# Autodesk Inventor assembly: Longhouse
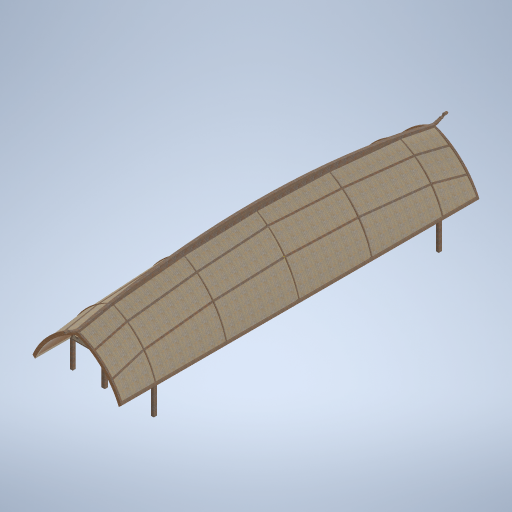
[picture p0: Inventor's stored thumbnail of the model, 512x512]
Saved by Autodesk Inventor 2024.2 (Build 282272000, 272)
## iProperties
Created: 2024-05-22
Part Number: Longhouse
Document SubType Name: Assembly
Designer: LOSTER_1
Author: LOSTER_1
## Documents named in this file (3)
- C:\Users\LOSTER_1\OneDrive\桌面\school\senior\Inventor_Project\Longhouse.iam
- C:\Users\LOSTER_1\OneDrive\桌面\school\senior\Inventor_Project\ROOF\Roof.iam
- C:\Users\LOSTER_1\OneDrive\桌面\school\senior\Inventor_Project\WALL\WallBody.iam
## Components (2 placed, 2 different names)
1. Roof:1 [sub-assembly] — Mate:1
2. WallBody:1 [sub-assembly] — Mate:1
## Relationships (1: Mate 1)
- Mate:1: Roof:1 ↔ WallBody:1
